# Autodesk Inventor assembly: wheeledArmDrop
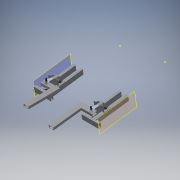
[picture p0: Inventor's stored thumbnail of the model, 180x180]
Saved by Autodesk Inventor 2016 (Build 200138000, 138)
## iProperties
Created: 2018-01-25
Part Number: wheeledArmDrop
Document SubType Name: Assembly
Designer: New User
Author: New User
## Documents named in this file (7)
- C:\Users\New User\Documents\Creations\2018\wheeledArmDrop.iam
- C:\Users\New User\Downloads\1_x_2_x_0_100_Pre-Drilled_VersaFrame_Aluminum_Tube_Stock_59_217-3453.ipt
- C:\Users\New User\Downloads\0_500_Hex_ID_x_1_125_OD_x_0_313_WD_Flanged_Bearing_v2_217-3875.ipt
- C:\Users\New User\Downloads\1_x_2_x_0_100_Pre-Drilled_VersaFrame_Aluminum_Tube_Stock_59_217-3453 (1).ipt
- C:\Users\New User\Downloads\1_2_Hex_x_0_201_ID_ThunderHex_Stock_18_217-4017.ipt
- C:\Users\New User\Downloads\VersaFrame_End_Bearing_Gusset_217-3554.ipt
- C:\Users\New User\Downloads\VersaFrame_Corner_Gusset_217-4238.ipt
## Components (40 placed, 6 different names)
1. 1_x_2_x_0_100_Pre-Drilled_VersaFrame_Aluminum_Tube_Stock_59_217-3453:1 — Flush:1, Mate:1, Flush:2, Flush:6, Mate:34, Mate:36, Mate:43, Flush:29
2. 1_x_2_x_0_100_Pre-Drilled_VersaFrame_Aluminum_Tube_Stock_59_217-3453:2 — Flush:1, Mate:1, Flush:2, Flush:9, Mate:32, Mate:33, Mate:42, Flush:13, Flush:14, Flush:24
3. 0_500_Hex_ID_x_1_125_OD_x_0_313_WD_Flanged_Bearing_v2_217-3875:2 — Mate:17, Mate:35
4. 0_500_Hex_ID_x_1_125_OD_x_0_313_WD_Flanged_Bearing_v2_217-3875:3 — Mate:18, Mate:31
5. 1_x_2_x_0_100_Pre-Drilled_VersaFrame_Aluminum_Tube_Stock_59_217-3453 (1):1 — Mate:12, Mate:13, Flush:7, Mate:14, Flush:9, Mate:20, Mate:21, Mate:22, Mate:23
6. 1_2_Hex_x_0_201_ID_ThunderHex_Stock_18_217-4017:1 — Flush:6, Flush:7, Mate:15, Mate:16, Mate:17, Mate:18
7. 0_500_Hex_ID_x_1_125_OD_x_0_313_WD_Flanged_Bearing_v2_217-3875:4 — Mate:12, Mate:14, Mate:15
8. 0_500_Hex_ID_x_1_125_OD_x_0_313_WD_Flanged_Bearing_v2_217-3875:5 — Mate:13, Mate:16
9. VersaFrame_End_Bearing_Gusset_217-3554:1 — Mate:20, Mate:24, Mate:25, Mate:27, Mate:29
10. VersaFrame_End_Bearing_Gusset_217-3554:2 — Mate:21, Mate:22, Mate:23, Mate:24, Mate:25, Mate:26, Mate:28, Flush:12
11. 0_500_Hex_ID_x_1_125_OD_x_0_313_WD_Flanged_Bearing_v2_217-3875:6 — Mate:26, Mate:28, Mate:30, Flush:10
12. 0_500_Hex_ID_x_1_125_OD_x_0_313_WD_Flanged_Bearing_v2_217-3875:7 — Mate:27, Mate:29
13. 1_2_Hex_x_0_201_ID_ThunderHex_Stock_18_217-4017:2 — Mate:30, Flush:10, Mate:37
14. VersaFrame_Corner_Gusset_217-4238:1 — Mate:34, Mate:35, Mate:36, Mate:43
15. VersaFrame_Corner_Gusset_217-4238:2 — Mate:31, Mate:32, Mate:33
16. 1_x_2_x_0_100_Pre-Drilled_VersaFrame_Aluminum_Tube_Stock_59_217-3453:3 — Mate:39, Flush:11, Mate:40, Mate:41, Flush:12, Mate:44, Flush:15, Flush:16
17. 0_500_Hex_ID_x_1_125_OD_x_0_313_WD_Flanged_Bearing_v2_217-3875:8 — Mate:37, Mate:38, Mate:41
18. 0_500_Hex_ID_x_1_125_OD_x_0_313_WD_Flanged_Bearing_v2_217-3875:9 — Mate:38, Mate:39, Flush:11, Mate:40
19. 1_x_2_x_0_100_Pre-Drilled_VersaFrame_Aluminum_Tube_Stock_59_217-3453:4 — Mate:42, Flush:13, Flush:14, Flush:27
20. 1_x_2_x_0_100_Pre-Drilled_VersaFrame_Aluminum_Tube_Stock_59_217-3453:5 — Mate:44, Flush:15, Flush:16
21. 1_x_2_x_0_100_Pre-Drilled_VersaFrame_Aluminum_Tube_Stock_59_217-3453:6 — Flush:24, Flush:25
22. 1_x_2_x_0_100_Pre-Drilled_VersaFrame_Aluminum_Tube_Stock_59_217-3453:7 — Flush:26, Mate:76, Flush:28
23. 0_500_Hex_ID_x_1_125_OD_x_0_313_WD_Flanged_Bearing_v2_217-3875:10 — Mate:75
24. 0_500_Hex_ID_x_1_125_OD_x_0_313_WD_Flanged_Bearing_v2_217-3875:11 — Mate:74
25. 1_x_2_x_0_100_Pre-Drilled_VersaFrame_Aluminum_Tube_Stock_59_217-3453 (1):2
26. 1_2_Hex_x_0_201_ID_ThunderHex_Stock_18_217-4017:3
27. 0_500_Hex_ID_x_1_125_OD_x_0_313_WD_Flanged_Bearing_v2_217-3875:12
28. 0_500_Hex_ID_x_1_125_OD_x_0_313_WD_Flanged_Bearing_v2_217-3875:13
29. VersaFrame_End_Bearing_Gusset_217-3554:3
30. VersaFrame_End_Bearing_Gusset_217-3554:4 — Flush:31
31. 0_500_Hex_ID_x_1_125_OD_x_0_313_WD_Flanged_Bearing_v2_217-3875:14
32. 0_500_Hex_ID_x_1_125_OD_x_0_313_WD_Flanged_Bearing_v2_217-3875:15
33. 1_2_Hex_x_0_201_ID_ThunderHex_Stock_18_217-4017:4
34. VersaFrame_Corner_Gusset_217-4238:3 — Mate:75
35. VersaFrame_Corner_Gusset_217-4238:4 — Mate:74
36. 0_500_Hex_ID_x_1_125_OD_x_0_313_WD_Flanged_Bearing_v2_217-3875:16 — Mate:79, Mate:80
37. 0_500_Hex_ID_x_1_125_OD_x_0_313_WD_Flanged_Bearing_v2_217-3875:17 — Mate:78, Flush:30
38. 1_x_2_x_0_100_Pre-Drilled_VersaFrame_Aluminum_Tube_Stock_59_217-3453:8 — Flush:25, Flush:26, Mate:76, Flush:27
39. 1_x_2_x_0_100_Pre-Drilled_VersaFrame_Aluminum_Tube_Stock_59_217-3453:9 — Mate:78, Flush:30, Mate:79, Mate:80, Flush:31, Flush:32, Mate:81, Flush:33
40. 1_x_2_x_0_100_Pre-Drilled_VersaFrame_Aluminum_Tube_Stock_59_217-3453:10 — Flush:32, Mate:81, Flush:33
## Relationships (97: Mate 69, Flush 28)
- Flush:1: 1_x_2_x_0_100_Pre-Drilled_VersaFrame_Aluminum_Tube_Stock_59_217-3453:1 ↔ 1_x_2_x_0_100_Pre-Drilled_VersaFrame_Aluminum_Tube_Stock_59_217-3453:2
- Mate:1 (50.8 mm): 1_x_2_x_0_100_Pre-Drilled_VersaFrame_Aluminum_Tube_Stock_59_217-3453:1 ↔ 1_x_2_x_0_100_Pre-Drilled_VersaFrame_Aluminum_Tube_Stock_59_217-3453:2
- Flush:2: 1_x_2_x_0_100_Pre-Drilled_VersaFrame_Aluminum_Tube_Stock_59_217-3453:1 ↔ 1_x_2_x_0_100_Pre-Drilled_VersaFrame_Aluminum_Tube_Stock_59_217-3453:2
- Flush:6: 1_x_2_x_0_100_Pre-Drilled_VersaFrame_Aluminum_Tube_Stock_59_217-3453:1 ↔ 1_2_Hex_x_0_201_ID_ThunderHex_Stock_18_217-4017:1
- Mate:12: 1_x_2_x_0_100_Pre-Drilled_VersaFrame_Aluminum_Tube_Stock_59_217-3453 (1):1 ↔ 0_500_Hex_ID_x_1_125_OD_x_0_313_WD_Flanged_Bearing_v2_217-3875:4
- Mate:13: 1_x_2_x_0_100_Pre-Drilled_VersaFrame_Aluminum_Tube_Stock_59_217-3453 (1):1 ↔ 0_500_Hex_ID_x_1_125_OD_x_0_313_WD_Flanged_Bearing_v2_217-3875:5
- Flush:7 (-22.86 mm): 1_x_2_x_0_100_Pre-Drilled_VersaFrame_Aluminum_Tube_Stock_59_217-3453 (1):1 ↔ 1_2_Hex_x_0_201_ID_ThunderHex_Stock_18_217-4017:1
- Mate:14 (-15.24 mm): 1_x_2_x_0_100_Pre-Drilled_VersaFrame_Aluminum_Tube_Stock_59_217-3453 (1):1 ↔ 0_500_Hex_ID_x_1_125_OD_x_0_313_WD_Flanged_Bearing_v2_217-3875:4
- Mate:15: 1_2_Hex_x_0_201_ID_ThunderHex_Stock_18_217-4017:1 ↔ 0_500_Hex_ID_x_1_125_OD_x_0_313_WD_Flanged_Bearing_v2_217-3875:4
- Mate:16: 1_2_Hex_x_0_201_ID_ThunderHex_Stock_18_217-4017:1 ↔ 0_500_Hex_ID_x_1_125_OD_x_0_313_WD_Flanged_Bearing_v2_217-3875:5
- Mate:17: 0_500_Hex_ID_x_1_125_OD_x_0_313_WD_Flanged_Bearing_v2_217-3875:2 ↔ 1_2_Hex_x_0_201_ID_ThunderHex_Stock_18_217-4017:1
- Mate:18: 0_500_Hex_ID_x_1_125_OD_x_0_313_WD_Flanged_Bearing_v2_217-3875:3 ↔ 1_2_Hex_x_0_201_ID_ThunderHex_Stock_18_217-4017:1
- Flush:9 (39.37 mm): 1_x_2_x_0_100_Pre-Drilled_VersaFrame_Aluminum_Tube_Stock_59_217-3453:2 ↔ 1_x_2_x_0_100_Pre-Drilled_VersaFrame_Aluminum_Tube_Stock_59_217-3453 (1):1
- Mate:20: 1_x_2_x_0_100_Pre-Drilled_VersaFrame_Aluminum_Tube_Stock_59_217-3453 (1):1 ↔ VersaFrame_End_Bearing_Gusset_217-3554:1
- Mate:21: 1_x_2_x_0_100_Pre-Drilled_VersaFrame_Aluminum_Tube_Stock_59_217-3453 (1):1 ↔ VersaFrame_End_Bearing_Gusset_217-3554:2
- Mate:22: 1_x_2_x_0_100_Pre-Drilled_VersaFrame_Aluminum_Tube_Stock_59_217-3453 (1):1 ↔ VersaFrame_End_Bearing_Gusset_217-3554:2
- Mate:23: 1_x_2_x_0_100_Pre-Drilled_VersaFrame_Aluminum_Tube_Stock_59_217-3453 (1):1 ↔ VersaFrame_End_Bearing_Gusset_217-3554:2
- Mate:24: VersaFrame_End_Bearing_Gusset_217-3554:1 ↔ VersaFrame_End_Bearing_Gusset_217-3554:2
- Mate:25: VersaFrame_End_Bearing_Gusset_217-3554:1 ↔ VersaFrame_End_Bearing_Gusset_217-3554:2
- Mate:26: VersaFrame_End_Bearing_Gusset_217-3554:2 ↔ 0_500_Hex_ID_x_1_125_OD_x_0_313_WD_Flanged_Bearing_v2_217-3875:6
- Mate:27: VersaFrame_End_Bearing_Gusset_217-3554:1 ↔ 0_500_Hex_ID_x_1_125_OD_x_0_313_WD_Flanged_Bearing_v2_217-3875:7
- Mate:28: VersaFrame_End_Bearing_Gusset_217-3554:2 ↔ 0_500_Hex_ID_x_1_125_OD_x_0_313_WD_Flanged_Bearing_v2_217-3875:6
- Mate:29: VersaFrame_End_Bearing_Gusset_217-3554:1 ↔ 0_500_Hex_ID_x_1_125_OD_x_0_313_WD_Flanged_Bearing_v2_217-3875:7
- Mate:30: 0_500_Hex_ID_x_1_125_OD_x_0_313_WD_Flanged_Bearing_v2_217-3875:6 ↔ 1_2_Hex_x_0_201_ID_ThunderHex_Stock_18_217-4017:2
- Flush:10 (-25.4 mm): 0_500_Hex_ID_x_1_125_OD_x_0_313_WD_Flanged_Bearing_v2_217-3875:6 ↔ 1_2_Hex_x_0_201_ID_ThunderHex_Stock_18_217-4017:2
- Mate:31: 0_500_Hex_ID_x_1_125_OD_x_0_313_WD_Flanged_Bearing_v2_217-3875:3 ↔ VersaFrame_Corner_Gusset_217-4238:2
- Mate:32: 1_x_2_x_0_100_Pre-Drilled_VersaFrame_Aluminum_Tube_Stock_59_217-3453:2 ↔ VersaFrame_Corner_Gusset_217-4238:2
- Mate:33: 1_x_2_x_0_100_Pre-Drilled_VersaFrame_Aluminum_Tube_Stock_59_217-3453:2 ↔ VersaFrame_Corner_Gusset_217-4238:2
- Mate:34: 1_x_2_x_0_100_Pre-Drilled_VersaFrame_Aluminum_Tube_Stock_59_217-3453:1 ↔ VersaFrame_Corner_Gusset_217-4238:1
- Mate:35: 0_500_Hex_ID_x_1_125_OD_x_0_313_WD_Flanged_Bearing_v2_217-3875:2 ↔ VersaFrame_Corner_Gusset_217-4238:1
- Mate:36: 1_x_2_x_0_100_Pre-Drilled_VersaFrame_Aluminum_Tube_Stock_59_217-3453:1 ↔ VersaFrame_Corner_Gusset_217-4238:1
- Mate:37: 1_2_Hex_x_0_201_ID_ThunderHex_Stock_18_217-4017:2 ↔ 0_500_Hex_ID_x_1_125_OD_x_0_313_WD_Flanged_Bearing_v2_217-3875:8
- Mate:38: 0_500_Hex_ID_x_1_125_OD_x_0_313_WD_Flanged_Bearing_v2_217-3875:8 ↔ 0_500_Hex_ID_x_1_125_OD_x_0_313_WD_Flanged_Bearing_v2_217-3875:9
- Mate:39: 1_x_2_x_0_100_Pre-Drilled_VersaFrame_Aluminum_Tube_Stock_59_217-3453:3 ↔ 0_500_Hex_ID_x_1_125_OD_x_0_313_WD_Flanged_Bearing_v2_217-3875:9
- Flush:11 (-38.1 mm): 1_x_2_x_0_100_Pre-Drilled_VersaFrame_Aluminum_Tube_Stock_59_217-3453:3 ↔ 0_500_Hex_ID_x_1_125_OD_x_0_313_WD_Flanged_Bearing_v2_217-3875:9
- Mate:40 (-25.4 mm): 1_x_2_x_0_100_Pre-Drilled_VersaFrame_Aluminum_Tube_Stock_59_217-3453:3 ↔ 0_500_Hex_ID_x_1_125_OD_x_0_313_WD_Flanged_Bearing_v2_217-3875:9
- Mate:41: 1_x_2_x_0_100_Pre-Drilled_VersaFrame_Aluminum_Tube_Stock_59_217-3453:3 ↔ 0_500_Hex_ID_x_1_125_OD_x_0_313_WD_Flanged_Bearing_v2_217-3875:8
- Flush:12 (15.24 mm): VersaFrame_End_Bearing_Gusset_217-3554:2 ↔ 1_x_2_x_0_100_Pre-Drilled_VersaFrame_Aluminum_Tube_Stock_59_217-3453:3
- Mate:42: 1_x_2_x_0_100_Pre-Drilled_VersaFrame_Aluminum_Tube_Stock_59_217-3453:2 ↔ 1_x_2_x_0_100_Pre-Drilled_VersaFrame_Aluminum_Tube_Stock_59_217-3453:4
- Flush:13: 1_x_2_x_0_100_Pre-Drilled_VersaFrame_Aluminum_Tube_Stock_59_217-3453:2 ↔ 1_x_2_x_0_100_Pre-Drilled_VersaFrame_Aluminum_Tube_Stock_59_217-3453:4
- Flush:14 (-25.4 mm): 1_x_2_x_0_100_Pre-Drilled_VersaFrame_Aluminum_Tube_Stock_59_217-3453:2 ↔ 1_x_2_x_0_100_Pre-Drilled_VersaFrame_Aluminum_Tube_Stock_59_217-3453:4
- Mate:43: 1_x_2_x_0_100_Pre-Drilled_VersaFrame_Aluminum_Tube_Stock_59_217-3453:1 ↔ VersaFrame_Corner_Gusset_217-4238:1
- Mate:44: 1_x_2_x_0_100_Pre-Drilled_VersaFrame_Aluminum_Tube_Stock_59_217-3453:3 ↔ 1_x_2_x_0_100_Pre-Drilled_VersaFrame_Aluminum_Tube_Stock_59_217-3453:5
- Flush:15: 1_x_2_x_0_100_Pre-Drilled_VersaFrame_Aluminum_Tube_Stock_59_217-3453:3 ↔ 1_x_2_x_0_100_Pre-Drilled_VersaFrame_Aluminum_Tube_Stock_59_217-3453:5
- Flush:16: 1_x_2_x_0_100_Pre-Drilled_VersaFrame_Aluminum_Tube_Stock_59_217-3453:3 ↔ 1_x_2_x_0_100_Pre-Drilled_VersaFrame_Aluminum_Tube_Stock_59_217-3453:5
- [Flush]: 1_x_2_x_0_100_Pre-Drilled_VersaFrame_Aluminum_Tube_Stock_59_217-3453:6 ↔ 1_x_2_x_0_100_Pre-Drilled_VersaFrame_Aluminum_Tube_Stock_59_217-3453:7
- [Mate] (50.8 mm): 1_x_2_x_0_100_Pre-Drilled_VersaFrame_Aluminum_Tube_Stock_59_217-3453:6 ↔ 1_x_2_x_0_100_Pre-Drilled_VersaFrame_Aluminum_Tube_Stock_59_217-3453:7
- [Flush]: 1_x_2_x_0_100_Pre-Drilled_VersaFrame_Aluminum_Tube_Stock_59_217-3453:6 ↔ 1_x_2_x_0_100_Pre-Drilled_VersaFrame_Aluminum_Tube_Stock_59_217-3453:7
- [Flush]: 1_x_2_x_0_100_Pre-Drilled_VersaFrame_Aluminum_Tube_Stock_59_217-3453:6 ↔ 1_2_Hex_x_0_201_ID_ThunderHex_Stock_18_217-4017:3
- [Mate]: 1_x_2_x_0_100_Pre-Drilled_VersaFrame_Aluminum_Tube_Stock_59_217-3453 (1):2 ↔ 0_500_Hex_ID_x_1_125_OD_x_0_313_WD_Flanged_Bearing_v2_217-3875:12
- [Mate]: 1_x_2_x_0_100_Pre-Drilled_VersaFrame_Aluminum_Tube_Stock_59_217-3453 (1):2 ↔ 0_500_Hex_ID_x_1_125_OD_x_0_313_WD_Flanged_Bearing_v2_217-3875:13
- [Flush] (-22.86 mm): 1_x_2_x_0_100_Pre-Drilled_VersaFrame_Aluminum_Tube_Stock_59_217-3453 (1):2 ↔ 1_2_Hex_x_0_201_ID_ThunderHex_Stock_18_217-4017:3
- [Mate] (-15.24 mm): 1_x_2_x_0_100_Pre-Drilled_VersaFrame_Aluminum_Tube_Stock_59_217-3453 (1):2 ↔ 0_500_Hex_ID_x_1_125_OD_x_0_313_WD_Flanged_Bearing_v2_217-3875:12
- [Mate]: 1_2_Hex_x_0_201_ID_ThunderHex_Stock_18_217-4017:3 ↔ 0_500_Hex_ID_x_1_125_OD_x_0_313_WD_Flanged_Bearing_v2_217-3875:12
- [Mate]: 1_2_Hex_x_0_201_ID_ThunderHex_Stock_18_217-4017:3 ↔ 0_500_Hex_ID_x_1_125_OD_x_0_313_WD_Flanged_Bearing_v2_217-3875:13
- [Mate]: 0_500_Hex_ID_x_1_125_OD_x_0_313_WD_Flanged_Bearing_v2_217-3875:10 ↔ 1_2_Hex_x_0_201_ID_ThunderHex_Stock_18_217-4017:3
- [Mate]: 0_500_Hex_ID_x_1_125_OD_x_0_313_WD_Flanged_Bearing_v2_217-3875:11 ↔ 1_2_Hex_x_0_201_ID_ThunderHex_Stock_18_217-4017:3
- [Flush] (39.37 mm): 1_x_2_x_0_100_Pre-Drilled_VersaFrame_Aluminum_Tube_Stock_59_217-3453:7 ↔ 1_x_2_x_0_100_Pre-Drilled_VersaFrame_Aluminum_Tube_Stock_59_217-3453 (1):2
- [Mate]: 1_x_2_x_0_100_Pre-Drilled_VersaFrame_Aluminum_Tube_Stock_59_217-3453 (1):2 ↔ VersaFrame_End_Bearing_Gusset_217-3554:3
- [Mate]: 1_x_2_x_0_100_Pre-Drilled_VersaFrame_Aluminum_Tube_Stock_59_217-3453 (1):2 ↔ VersaFrame_End_Bearing_Gusset_217-3554:4
- [Mate]: 1_x_2_x_0_100_Pre-Drilled_VersaFrame_Aluminum_Tube_Stock_59_217-3453 (1):2 ↔ VersaFrame_End_Bearing_Gusset_217-3554:4
- [Mate]: 1_x_2_x_0_100_Pre-Drilled_VersaFrame_Aluminum_Tube_Stock_59_217-3453 (1):2 ↔ VersaFrame_End_Bearing_Gusset_217-3554:4
- [Mate]: VersaFrame_End_Bearing_Gusset_217-3554:3 ↔ VersaFrame_End_Bearing_Gusset_217-3554:4
- [Mate]: VersaFrame_End_Bearing_Gusset_217-3554:3 ↔ VersaFrame_End_Bearing_Gusset_217-3554:4
- [Mate]: VersaFrame_End_Bearing_Gusset_217-3554:4 ↔ 0_500_Hex_ID_x_1_125_OD_x_0_313_WD_Flanged_Bearing_v2_217-3875:14
- [Mate]: VersaFrame_End_Bearing_Gusset_217-3554:3 ↔ 0_500_Hex_ID_x_1_125_OD_x_0_313_WD_Flanged_Bearing_v2_217-3875:15
- [Mate]: VersaFrame_End_Bearing_Gusset_217-3554:4 ↔ 0_500_Hex_ID_x_1_125_OD_x_0_313_WD_Flanged_Bearing_v2_217-3875:14
- [Mate]: VersaFrame_End_Bearing_Gusset_217-3554:3 ↔ 0_500_Hex_ID_x_1_125_OD_x_0_313_WD_Flanged_Bearing_v2_217-3875:15
- [Mate]: 0_500_Hex_ID_x_1_125_OD_x_0_313_WD_Flanged_Bearing_v2_217-3875:14 ↔ 1_2_Hex_x_0_201_ID_ThunderHex_Stock_18_217-4017:4
- [Flush] (-25.4 mm): 0_500_Hex_ID_x_1_125_OD_x_0_313_WD_Flanged_Bearing_v2_217-3875:14 ↔ 1_2_Hex_x_0_201_ID_ThunderHex_Stock_18_217-4017:4
- [Mate]: 0_500_Hex_ID_x_1_125_OD_x_0_313_WD_Flanged_Bearing_v2_217-3875:11 ↔ VersaFrame_Corner_Gusset_217-4238:4
- [Mate]: 1_x_2_x_0_100_Pre-Drilled_VersaFrame_Aluminum_Tube_Stock_59_217-3453:7 ↔ VersaFrame_Corner_Gusset_217-4238:4
- [Mate]: 1_x_2_x_0_100_Pre-Drilled_VersaFrame_Aluminum_Tube_Stock_59_217-3453:7 ↔ VersaFrame_Corner_Gusset_217-4238:4
- [Mate]: 1_x_2_x_0_100_Pre-Drilled_VersaFrame_Aluminum_Tube_Stock_59_217-3453:6 ↔ VersaFrame_Corner_Gusset_217-4238:3
- [Mate]: 0_500_Hex_ID_x_1_125_OD_x_0_313_WD_Flanged_Bearing_v2_217-3875:10 ↔ VersaFrame_Corner_Gusset_217-4238:3
- [Mate]: 1_x_2_x_0_100_Pre-Drilled_VersaFrame_Aluminum_Tube_Stock_59_217-3453:6 ↔ VersaFrame_Corner_Gusset_217-4238:3
- [Mate]: 1_2_Hex_x_0_201_ID_ThunderHex_Stock_18_217-4017:4 ↔ 0_500_Hex_ID_x_1_125_OD_x_0_313_WD_Flanged_Bearing_v2_217-3875:16
- [Mate]: 0_500_Hex_ID_x_1_125_OD_x_0_313_WD_Flanged_Bearing_v2_217-3875:16 ↔ 0_500_Hex_ID_x_1_125_OD_x_0_313_WD_Flanged_Bearing_v2_217-3875:17
- [Mate]: 1_x_2_x_0_100_Pre-Drilled_VersaFrame_Aluminum_Tube_Stock_59_217-3453:6 ↔ VersaFrame_Corner_Gusset_217-4238:3
- Flush:24: 1_x_2_x_0_100_Pre-Drilled_VersaFrame_Aluminum_Tube_Stock_59_217-3453:2 ↔ 1_x_2_x_0_100_Pre-Drilled_VersaFrame_Aluminum_Tube_Stock_59_217-3453:6
- Mate:74: 0_500_Hex_ID_x_1_125_OD_x_0_313_WD_Flanged_Bearing_v2_217-3875:11 ↔ VersaFrame_Corner_Gusset_217-4238:4
- Mate:75: 0_500_Hex_ID_x_1_125_OD_x_0_313_WD_Flanged_Bearing_v2_217-3875:10 ↔ VersaFrame_Corner_Gusset_217-4238:3
- Flush:25: 1_x_2_x_0_100_Pre-Drilled_VersaFrame_Aluminum_Tube_Stock_59_217-3453:6 ↔ 1_x_2_x_0_100_Pre-Drilled_VersaFrame_Aluminum_Tube_Stock_59_217-3453:8
- Flush:26 (-50.8 mm): 1_x_2_x_0_100_Pre-Drilled_VersaFrame_Aluminum_Tube_Stock_59_217-3453:7 ↔ 1_x_2_x_0_100_Pre-Drilled_VersaFrame_Aluminum_Tube_Stock_59_217-3453:8
- Mate:76: 1_x_2_x_0_100_Pre-Drilled_VersaFrame_Aluminum_Tube_Stock_59_217-3453:7 ↔ 1_x_2_x_0_100_Pre-Drilled_VersaFrame_Aluminum_Tube_Stock_59_217-3453:8
- Flush:27: 1_x_2_x_0_100_Pre-Drilled_VersaFrame_Aluminum_Tube_Stock_59_217-3453:4 ↔ 1_x_2_x_0_100_Pre-Drilled_VersaFrame_Aluminum_Tube_Stock_59_217-3453:8
- Flush:28 (50.8 mm): 1_x_2_x_0_100_Pre-Drilled_VersaFrame_Aluminum_Tube_Stock_59_217-3453:7
- Flush:29 (50.8 mm): 1_x_2_x_0_100_Pre-Drilled_VersaFrame_Aluminum_Tube_Stock_59_217-3453:1
- Mate:77 (-685.8 mm)
- Mate:78: 0_500_Hex_ID_x_1_125_OD_x_0_313_WD_Flanged_Bearing_v2_217-3875:17 ↔ 1_x_2_x_0_100_Pre-Drilled_VersaFrame_Aluminum_Tube_Stock_59_217-3453:9
- Flush:30 (38.1 mm): 0_500_Hex_ID_x_1_125_OD_x_0_313_WD_Flanged_Bearing_v2_217-3875:17 ↔ 1_x_2_x_0_100_Pre-Drilled_VersaFrame_Aluminum_Tube_Stock_59_217-3453:9
- Mate:79 (-15.24 mm): 0_500_Hex_ID_x_1_125_OD_x_0_313_WD_Flanged_Bearing_v2_217-3875:16 ↔ 1_x_2_x_0_100_Pre-Drilled_VersaFrame_Aluminum_Tube_Stock_59_217-3453:9
- Mate:80: 0_500_Hex_ID_x_1_125_OD_x_0_313_WD_Flanged_Bearing_v2_217-3875:16 ↔ 1_x_2_x_0_100_Pre-Drilled_VersaFrame_Aluminum_Tube_Stock_59_217-3453:9
- Flush:31 (15.24 mm): VersaFrame_End_Bearing_Gusset_217-3554:4 ↔ 1_x_2_x_0_100_Pre-Drilled_VersaFrame_Aluminum_Tube_Stock_59_217-3453:9
- Flush:32: 1_x_2_x_0_100_Pre-Drilled_VersaFrame_Aluminum_Tube_Stock_59_217-3453:9 ↔ 1_x_2_x_0_100_Pre-Drilled_VersaFrame_Aluminum_Tube_Stock_59_217-3453:10
- Mate:81: 1_x_2_x_0_100_Pre-Drilled_VersaFrame_Aluminum_Tube_Stock_59_217-3453:9 ↔ 1_x_2_x_0_100_Pre-Drilled_VersaFrame_Aluminum_Tube_Stock_59_217-3453:10
- Flush:33: 1_x_2_x_0_100_Pre-Drilled_VersaFrame_Aluminum_Tube_Stock_59_217-3453:9 ↔ 1_x_2_x_0_100_Pre-Drilled_VersaFrame_Aluminum_Tube_Stock_59_217-3453:10
## Named parameters: d68_d46 = 0 mm, d69_d47 = 0 mm, d70_d48 = 0 mm, d71_d49 = 0 mm, d72_d50 = 0 mm, d73_d33 = 0 mm, d74_d34 = 0 mm, d75_d35 = 0 mm, d76_d36 = 0 mm, d77_d37 = 0 mm, d78_d38 = 0 mm, d79_d39 = 0 mm, d80_d40 = 0 mm, d81_d41 = 0 mm, d82_d42 = -25.4 mm, d83_d43 = 0 mm, d84_d44 = 0 mm, d85_d45 = 0 mm, d86_d24 = -15.24 mm, d87_d25 = 0 mm, d88_d26 = 0 mm, d89_d27 = 0 mm, d90_d28 = 0 mm, d91_d30 = 39.37 mm, d92_d31 = 0 mm, d93_d32 = 0 mm, d94_d17 = 0 mm, d95_d20 = 0 mm, d96_d21 = 0 mm, d97_d22 = -22.86 mm, d98_d63 = 0 mm, d99_d1 = 50.8 mm, d100_d2 = 0 mm, d101_d0 = 0 mm
